# Autodesk Inventor assembly: bottom
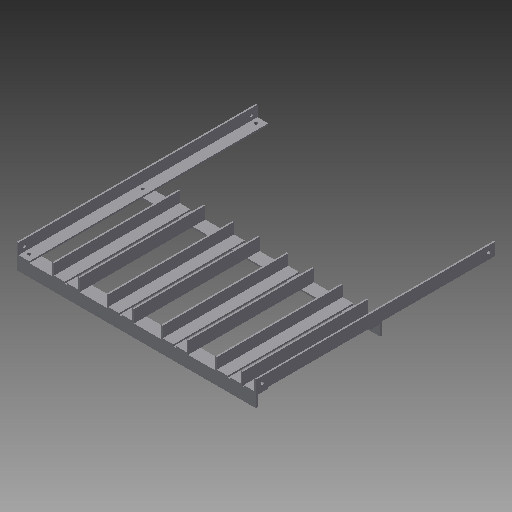
[picture p0: Inventor's stored thumbnail of the model, 512x512]
Saved by Autodesk Inventor 2017 (Build 210142000, 142)
## iProperties
Created: 2018-10-22
Part Number: bottom
Document SubType Name: Assembly
Designer: ddeboer
Author: ddeboer
## Documents named in this file (3)
- C:\Users\ddeboer\Desktop\snap_holder\bottom.iam
- C:\Users\ddeboer\Desktop\snap_holder\ladder.iam
- C:\Users\ddeboer\Desktop\snap_holder\angle_L11.ipt
## Components (3 placed, 3 different names)
1. ladder:1 [sub-assembly] — Insert:1, Flush:1, Insert:2, Flush:2
2. angle_L11:left — Insert:1, Flush:1
3. angle_L11:right — Insert:2, Flush:2
## Relationships (4: Insert 2, Flush 2)
- Insert:1: ladder:1 ↔ angle_L11:left
- Flush:1: ladder:1 ↔ angle_L11:left
- Insert:2: ladder:1 ↔ angle_L11:right
- Flush:2: ladder:1 ↔ angle_L11:right
